# Autodesk Inventor assembly: Electric Box
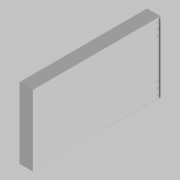
[picture p0: Inventor's stored thumbnail of the model, 180x180]
Saved by Autodesk Inventor 2020 (Build 240168000, 168)
## iProperties
Created: 2020-08-05
Part Number: Electric Box
Document SubType Name: Assembly
Designer: Abbas
Author: Abbas
## Documents named in this file (4)
- C:\Users\LENOVO\Desktop\Graduation Project\Fish Farming Unit\Electric Box\Electric Box.iam
- C:\Users\LENOVO\Desktop\Graduation Project\Fish Farming Unit\Electric Box\Electric Box.ipt
- C:\Users\LENOVO\Desktop\Graduation Project\Fish Farming Unit\Electric Box\Peice 1.ipt
- C:\Users\LENOVO\Desktop\Graduation Project\Fish Farming Unit\Electric Box\Front Assamblied.iam
## Components (4 placed, 3 different names)
1. Electric Box:2 — Mate:1, Insert:1, Mate:2, Insert:2
2. Peice 1:1 — Mate:1, Insert:1, Insert:3
3. Peice 1:2 — Mate:2, Insert:2
4. Front Assamblied:1 [sub-assembly] — Insert:3
## Relationships (5: Insert 3, Mate 2)
- Mate:1: Electric Box:2 ↔ Peice 1:1
- Insert:1: Electric Box:2 ↔ Peice 1:1
- Mate:2: Electric Box:2 ↔ Peice 1:2
- Insert:2: Electric Box:2 ↔ Peice 1:2
- Insert:3: Peice 1:1 ↔ Front Assamblied:1
